# Autodesk Inventor assembly: GearMotor_Wheel
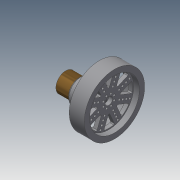
[picture p0: Inventor's stored thumbnail of the model, 180x180]
Saved by Autodesk Inventor 2014 SP1 (Build 180222100, 222)
## iProperties
Created: 2014-04-02
Part Number: GearMotor_Wheel
Document SubType Name: Assembly
Designer: tom
Author: tom
## Documents named in this file (5)
- C:\Users\tom\Documents\GitHub\Vacubot\Inventor\GearMotor_Wheel.iam
- C:\Users\tom\Documents\GitHub\Vacubot\Inventor\Motor Mount.ipt
- C:\Users\tom\Documents\GitHub\Vacubot\Inventor\Drive Motor.ipt
- C:\Users\tom\Documents\GitHub\Vacubot\Inventor\Clamping Hub.ipt
- C:\Users\tom\Documents\GitHub\Vacubot\Inventor\Wheel.ipt
## Components (4 placed, 4 different names)
1. Motor Mount:1
2. Drive Motor:1
3. Clamping Hub:1
4. Drive Wheel
## Relationships (6: Mate 5, Flush 1)
- [Mate]: Motor Mount:1 ↔ Drive Motor:1
- [Flush] (-5 mm): Motor Mount:1 ↔ Drive Motor:1
- [Mate]: Drive Motor:1 ↔ Clamping Hub:1
- [Mate]: Drive Motor:1 ↔ Clamping Hub:1
- [Mate]: Clamping Hub:1 ↔ Drive Wheel
- [Mate]: Clamping Hub:1 ↔ Drive Wheel
